# Autodesk Inventor assembly: lower_leg_link
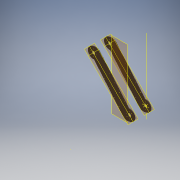
[picture p0: Inventor's stored thumbnail of the model, 180x180]
Saved by Autodesk Inventor 2018 (Build 220112000, 112)
## iProperties
Created: 2018-11-30
Part Number: lower_leg_link
Document SubType Name: Assembly
Designer: bitbots
Author: bitbots
## Documents named in this file (2)
- C:\Users\jaspe\bitbots_hardware\wolfgang\assembly\legs\lower_leg_link.iam
- C:\Users\jaspe\bitbots_hardware\wolfgang\assembly\legs\lower_leg_MIR.ipt
## Components (2 placed, 1 different names)
1. lower_leg_MIR:1 — Mate:1, Angle:1, Mate:2, Mate:4, Mate:5, Mate:9, Mate:10, Symmetry:1, Mate:12, Mate:13
2. lower_leg_MIR:2 — Mate:1, Angle:1, Mate:2, Symmetry:1, Mate:17, Mate:18
## Relationships (18: Mate 16, Angle 1, Symmetry 1)
- Mate:1 (51.9 mm): lower_leg_MIR:1 ↔ lower_leg_MIR:2
- Angle:1 (0 deg): lower_leg_MIR:1 ↔ lower_leg_MIR:2
- Mate:2: lower_leg_MIR:1 ↔ lower_leg_MIR:2
- Mate:4: lower_leg_MIR:1
- Mate:5: lower_leg_MIR:1
- Mate:6
- Mate:7
- Mate:9: lower_leg_MIR:1
- Mate:10: lower_leg_MIR:1
- Symmetry:1: lower_leg_MIR:1 ↔ lower_leg_MIR:2
- Mate:11
- Mate:12: lower_leg_MIR:1
- Mate:13: lower_leg_MIR:1
- Mate:14
- Mate:15
- Mate:16
- Mate:17: lower_leg_MIR:2
- Mate:18: lower_leg_MIR:2
